# Autodesk Inventor assembly: Lifting Mechanism
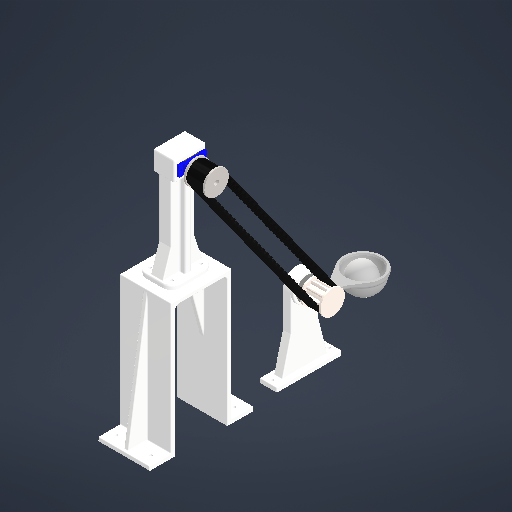
[picture p0: Inventor's stored thumbnail of the model, 512x512]
Saved by Autodesk Inventor 2026.2 (Build 302298010, 298A)
## iProperties
Created: 2026-05-22
Part Number: Lifting Mechanism
Description: STEP AP214
Document SubType Name: Assembly
Designer: lenovo
Sending System: SolidWorks 2025
Preprocessor: SwSTEP 2.0
Title: Lifting Mechanism.STEP
Revision Number: Symmetric
## Documents named in this file (11)
- C:\Users\lenovo\Downloads\STEP-20260522T230805Z-3-001\STEP\Lifting Mechanism\Lifting Mechanism\Lifting Mechanism.iam
- C:\Users\lenovo\Downloads\STEP-20260522T230805Z-3-001\STEP\Lifting Mechanism\Lifting Mechanism\SG90 - Micro Servo 9g - Tower Pro.1_Peça.ipt
- C:\Users\lenovo\Downloads\STEP-20260522T230805Z-3-001\STEP\Lifting Mechanism\Lifting Mechanism\NSK_6000ZZ.iam
- C:\Users\lenovo\Downloads\STEP-20260522T230805Z-3-001\STEP\Lifting Mechanism\Lifting Mechanism\Conveyor Gear_DIN - Spur gear 2M 10T 14.5PA 20FW ---S10A75H50L5N.ipt
- C:\Users\lenovo\Downloads\STEP-20260522T230805Z-3-001\STEP\Lifting Mechanism\Lifting Mechanism\Plummer Block.ipt
- C:\Users\lenovo\Downloads\STEP-20260522T230805Z-3-001\STEP\Lifting Mechanism\Lifting Mechanism\Servo Gear_DIN - Spur gear 2M 10T 14.5PA 20FW ---S10A75H50L5N.ipt
- C:\Users\lenovo\Downloads\STEP-20260522T230805Z-3-001\STEP\Lifting Mechanism\Lifting Mechanism\Ball Holder.ipt
- C:\Users\lenovo\Downloads\STEP-20260522T230805Z-3-001\STEP\Lifting Mechanism\Lifting Mechanism\elevator.ipt
- C:\Users\lenovo\Downloads\STEP-20260522T230805Z-3-001\STEP\Lifting Mechanism\Lifting Mechanism\Conveyor Belt.ipt
- C:\Users\lenovo\Downloads\STEP-20260522T230805Z-3-001\STEP\Lifting Mechanism\Lifting Mechanism\N Stand.ipt
- F:\Semester 4\Basics of Mechatronics\Project\Small Ball.ipt
## Components (10 placed, 10 different names)
1. SG90 - Micro Servo 9g - Tower Pro.1_Peça_18 — Mate:2, Mate:12, Mate:13, Mate:14
2. NSK_6000ZZ_19 [sub-assembly] — Mate:5, Mate:6
3. Conveyor Gear_DIN - Spur gear 2M 10T 14.5PA 20FW ---S10A75H50L5N_21 — Mate:3, Mate:4
4. Plummer Block_22 — Mate:4, Mate:5, Mate:6
5. Servo Gear_DIN - Spur gear 2M 10T 14.5PA 20FW ---S10A75H50L5N_23 — Mate:1, Mate:2
6. Ball Holder_24 — Mate:15, Tangent:1
7. elevator_25 — Mate:8, Mate:9, Mate:10
8. Conveyor Belt_26 — Mate:1, Mate:3, Mate:15
9. N Stand_27 — Mate:8, Mate:9, Mate:10, Mate:12, Mate:13, Mate:14
10. Small Ball:1 — Tangent:1
## Relationships (14: Mate 13, Tangent 1)
- Mate:1: Servo Gear_DIN - Spur gear 2M 10T 14.5PA 20FW ---S10A75H50L5N_23 ↔ Conveyor Belt_26
- Mate:2: SG90 - Micro Servo 9g - Tower Pro.1_Peça_18 ↔ Servo Gear_DIN - Spur gear 2M 10T 14.5PA 20FW ---S10A75H50L5N_23
- Mate:3: Conveyor Gear_DIN - Spur gear 2M 10T 14.5PA 20FW ---S10A75H50L5N_21 ↔ Conveyor Belt_26
- Mate:4: Conveyor Gear_DIN - Spur gear 2M 10T 14.5PA 20FW ---S10A75H50L5N_21 ↔ Plummer Block_22
- Mate:5: NSK_6000ZZ_19 ↔ Plummer Block_22
- Mate:6: NSK_6000ZZ_19 ↔ Plummer Block_22
- Mate:8: elevator_25 ↔ N Stand_27
- Mate:9: elevator_25 ↔ N Stand_27
- Mate:10: elevator_25 ↔ N Stand_27
- Mate:12: SG90 - Micro Servo 9g - Tower Pro.1_Peça_18 ↔ N Stand_27
- Mate:13: SG90 - Micro Servo 9g - Tower Pro.1_Peça_18 ↔ N Stand_27
- Mate:14: SG90 - Micro Servo 9g - Tower Pro.1_Peça_18 ↔ N Stand_27
- Mate:15: Ball Holder_24 ↔ Conveyor Belt_26
- Tangent:1: Ball Holder_24 ↔ Small Ball:1
